# Autodesk Inventor assembly: Infinity
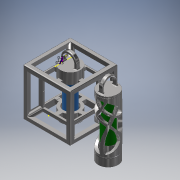
[picture p0: Inventor's stored thumbnail of the model, 180x180]
Saved by Autodesk Inventor 2019 (Build 230136000, 136)
## iProperties
Created: 2019-05-03
Part Number: Infinity
Document SubType Name: Assembly
Designer: Jorian Brusind
Author: Jorian Brusind
## Documents named in this file (3)
- C:\Users\Jorian Brusind\Documents\GitHub\PersonalProjects\Inventor Projects\Infinity\Infinity.iam
- C:\Users\Jorian Brusind\Documents\GitHub\PersonalProjects\Inventor Projects\Infinity\Time.iam
- C:\Users\Jorian Brusind\Documents\GitHub\PersonalProjects\Inventor Projects\Infinity\Space.iam
## Components (2 placed, 2 different names)
1. Time:1 [sub-assembly] — Flush:1, Flush:2
2. Space:1 [sub-assembly] — Flush:1, Flush:2
## Relationships (2: Flush 2)
- Flush:1: Time:1 ↔ Space:1
- Flush:2: Time:1 ↔ Space:1
